# Autodesk Inventor assembly: 22
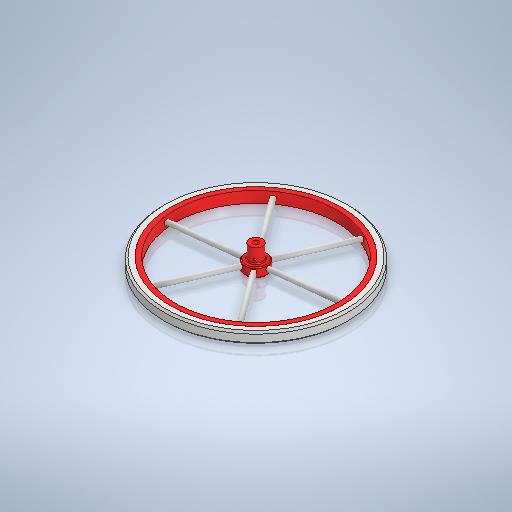
[picture p0: Inventor's stored thumbnail of the model, 512x512]
Saved by Autodesk Inventor 2025.1 (Build 291241000, 241)
## iProperties
Created: 2024-09-13
Part Number: 22
Document SubType Name: Assembly
Designer: ffogue
Author: ffogue
## Documents named in this file (5)
- C:\Users\ffogue\Documents\Inventor\Single cylinder Steam Engine\22.iam
- C:\Users\ffogue\Documents\Inventor\Single cylinder Steam Engine\22.1.ipt
- C:\Users\ffogue\Documents\Inventor\Single cylinder Steam Engine\22.3.ipt
- C:\Users\ffogue\Documents\Inventor\Single cylinder Steam Engine\22.2.ipt
- C:\Users\ffogue\Documents\Inventor\Single cylinder Steam Engine\22.4.ipt
## Components (9 placed, 4 different names)
1. 22.1:1 — Mate:2, Flush:1
2. 22.3:1 — Mate:1, Rotational:1, Mate:2, Flush:1, Mate:5
3. 22.4:1 — Mate:3, Mate:4
4. 22.2:1 — Mate:1, Rotational:1, Mate:3
5. 22.2:2
6. 22.2:3
7. 22.2:4
8. 22.2:5
9. 22.2:6
## Component patterns: (6 elements, first: 22.2:1)
## Relationships (8: Mate 6, RevoluteJoint 1, Flush 1)
- Mate:1: 22.3:1 ↔ 22.2:1
- Rotational:1 [RevoluteJoint] (-5 mm): 22.3:1 ↔ 22.2:1
- Mate:2: 22.1:1 ↔ 22.3:1
- Flush:1: 22.1:1 ↔ 22.3:1
- Mate:3: 22.4:1 ↔ 22.2:1
- Mate:4: 22.4:1
- Mate:5: 22.3:1
- Mate:6
